# Autodesk Inventor assembly: I_Przegub_final
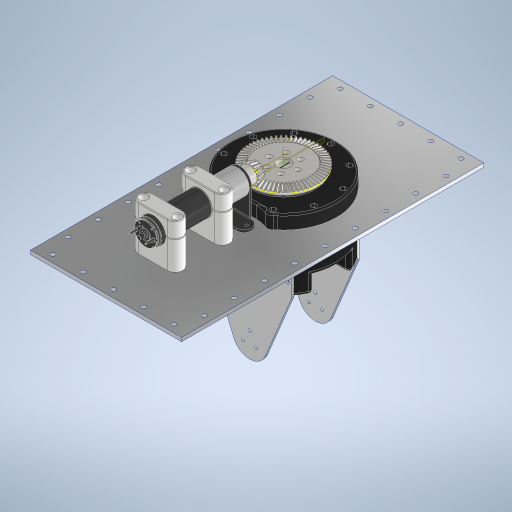
[picture p0: Inventor's stored thumbnail of the model, 512x512]
Saved by Autodesk Inventor 2023 (Build 270158000, 158)
## iProperties
Created: 2023-01-03
Part Number: I_Przegub_final
Document SubType Name: Assembly
Designer: komputer
Mass: 2476.88 g
Surface Area: 4078.03 cm^2
Volume: 1218.54 cm^3
Density: 2.03265 g/cm^3
Author: komputer
## Documents named in this file (12)
- C:\Users\Kamil\Desktop\KONARM\Konarm_1_przegub_final\I_Przegub_final.iam
- C:\Users\Kamil\Desktop\KONARM\Konarm_1_przegub_final\Assembly3\Design Accelerator\Bevel Gears1.iam
- C:\Users\Kamil\Desktop\KONARM\Konarm_1_przegub_final\32010-X-GY-002.ipt
- C:\Users\Kamil\Desktop\KONARM\Konarm_1_przegub_final\Podstawa.ipt
- C:\Users\Kamil\Desktop\KONARM\Konarm_1_przegub_final\podst.ipt
- C:\Users\Kamil\Desktop\KONARM\Konarm_1_przegub_final\Góra.ipt
- C:\Users\Kamil\Desktop\KONARM\Konarm_1_przegub_final\Uchwyt_silnika_1.ipt
- C:\Users\Kamil\Desktop\KONARM\Konarm_1_przegub_final\Uchwyt_silnika_2_dół.ipt
- C:\Users\Kamil\Desktop\KONARM\Konarm_1_przegub_final\Uchwyt_silnika_2_góra.ipt
- C:\Users\Kamil\Desktop\KONARM\Konarm_1_przegub_final\Faulhaber 3272G012C R.ipt
- C:\Users\Kamil\Desktop\KONARM\Konarm_1_przegub_final\lacznik.ipt
- C:\Users\Kamil\Desktop\KONARM\Konarm_1_przegub_final\BLACHA_2_Przegub.ipt
## Components (15 placed, 11 different names)
1. Bevel Gears:1 [sub-assembly] — Mate:1, Mate:2, Mate:4, Mate:8, Mate:15, Mate:16, Mate:34
2. 32010-X-GY-002:1 — Mate:1, Mate:2, Mate:3
3. Podstawa:1 — Mate:3, Mate:4, Mate:7, Mate:9, Mate:21, Mate:23, Mate:31, Mate:32
4. podst:1 — Mate:7, Mate:8, Mate:9, Zestawiające:64
5. Góra:1 — Mate:33, Mate:34, Równoległe:1, Zestawiające:38, Zestawiające:64, Zestawiające:65
6. Uchwyt_silnika_1:1 — Mate:15, Mate:16, Mate:29, Mate:30
7. Uchwyt_silnika_2_dół:1 — Mate:21, Mate:27
8. Uchwyt_silnika_2_dół:2 — Mate:23, Mate:26
9. Uchwyt_silnika_2_góra:1 — Mate:27
10. Uchwyt_silnika_2_góra:2 — Mate:26, Mate:28
11. Faulhaber 3272G012C R:1 — Mate:28, Mate:29, Mate:30
12. 32010-X-GY-002:2 — Mate:31, Mate:32, Mate:33, Zestawiające:38
13. lacznik:1 — Równoległe:1, Zestawiające:39, Zestawiające:40, Zestawiające:41, Zestawiające:42, Zestawiające:43, Zestawiające:44, Zestawiające:65
14. BLACHA_2_Przegub:1 — Zestawiające:39, Zestawiające:40, Zestawiające:41
15. BLACHA_2_Przegub:2 — Zestawiające:42, Zestawiające:43, Zestawiające:44
## Relationships (30: Mate 29, Flush 1)
- Mate:1 (0.5 mm): Bevel Gears:1 ↔ 32010-X-GY-002:1
- Mate:2: Bevel Gears:1 ↔ 32010-X-GY-002:1
- Mate:3 (0.5 mm): 32010-X-GY-002:1 ↔ Podstawa:1
- Mate:4: Bevel Gears:1 ↔ Podstawa:1
- Mate:7: Podstawa:1 ↔ podst:1
- Mate:8: Bevel Gears:1 ↔ podst:1
- Mate:9: Podstawa:1 ↔ podst:1
- Mate:15 (0.5 mm): Bevel Gears:1 ↔ Uchwyt_silnika_1:1
- Mate:16: Bevel Gears:1 ↔ Uchwyt_silnika_1:1
- Mate:21: Podstawa:1 ↔ Uchwyt_silnika_2_dół:1
- Mate:23: Podstawa:1 ↔ Uchwyt_silnika_2_dół:2
- Mate:26: Uchwyt_silnika_2_dół:2 ↔ Uchwyt_silnika_2_góra:2
- Mate:27: Uchwyt_silnika_2_dół:1 ↔ Uchwyt_silnika_2_góra:1
- Mate:28: Uchwyt_silnika_2_góra:2 ↔ Faulhaber 3272G012C R:1
- Mate:29: Uchwyt_silnika_1:1 ↔ Faulhaber 3272G012C R:1
- Mate:30: Uchwyt_silnika_1:1 ↔ Faulhaber 3272G012C R:1
- Mate:31: Podstawa:1 ↔ 32010-X-GY-002:2
- Mate:32: Podstawa:1 ↔ 32010-X-GY-002:2
- Mate:33 (0.3 mm): Góra:1 ↔ 32010-X-GY-002:2
- Mate:34: Bevel Gears:1 ↔ Góra:1
- Równoległe:1 [Flush]: Góra:1 ↔ lacznik:1
- Zestawiające:38 [Mate]: Góra:1 ↔ 32010-X-GY-002:2
- Zestawiające:39 [Mate]: lacznik:1 ↔ BLACHA_2_Przegub:1
- Zestawiające:40 [Mate]: lacznik:1 ↔ BLACHA_2_Przegub:1
- Zestawiające:41 [Mate]: lacznik:1 ↔ BLACHA_2_Przegub:1
- Zestawiające:42 [Mate]: lacznik:1 ↔ BLACHA_2_Przegub:2
- Zestawiające:43 [Mate]: lacznik:1 ↔ BLACHA_2_Przegub:2
- Zestawiające:44 [Mate]: lacznik:1 ↔ BLACHA_2_Przegub:2
- Zestawiające:64 [Mate] (8.1 mm): podst:1 ↔ Góra:1
- Zestawiające:65 [Mate]: Góra:1 ↔ lacznik:1
